# Autodesk Inventor assembly: PortaPiezas
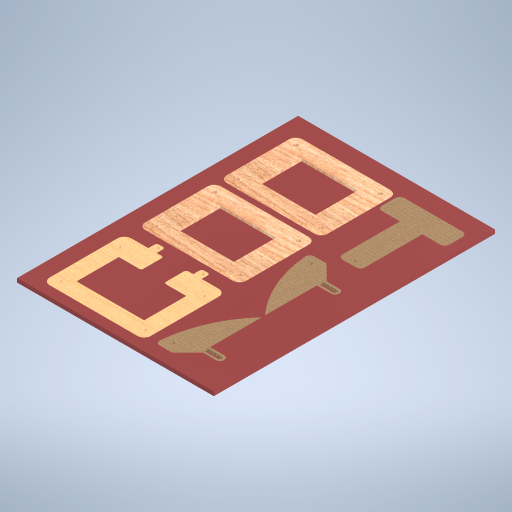
[picture p0: Inventor's stored thumbnail of the model, 512x512]
Saved by Autodesk Inventor 2023.1 (Build 271208000, 208)
## iProperties
Created: 2022-11-11
Part Number: PortaPiezas
Document SubType Name: Assembly
Designer: Daniel Peña
Author: Daniel Peña
## Documents named in this file (8)
- C:\Users\danie\Documents\UN\ProyectoRobotica\CAD\V3 - BigChungus\PortaPiezas.iam
- C:\Users\danie\Documents\UN\ProyectoRobotica\CAD\V3 - BigChungus\Base.ipt
- C:\Users\danie\Documents\UN\ProyectoRobotica\CAD\V3 - BigChungus\MarcoRompecabezas.ipt
- C:\Users\danie\Documents\UN\ProyectoRobotica\CAD\V3 - BigChungus\MarcoBC.ipt
- C:\Users\danie\Documents\UN\ProyectoRobotica\CAD\V3 - BigChungus\PistonBC.ipt
- C:\Users\danie\Documents\UN\ProyectoRobotica\CAD\V3 - BigChungus\TapaBC.ipt
- C:\Users\danie\Documents\UN\ProyectoRobotica\CAD\V3 - BigChungus\Dedo-BC.ipt
- C:\Users\danie\Documents\UN\ProyectoRobotica\CAD\PortaHerramienta\Ventosa.ipt
## Components (9 placed, 7 different names)
1. Base:1 — Flush:1, Mate:13, Mate:14, Mate:15, Mate:16, Mate:17, Mate:18, Flush:2, Flush:3
2. MarcoRompecabezas:1 — Flush:1, Mate:19, Flush:2, Flush:3, Mate:20, Mate:21, Mate:22, Mate:23, Mate:24, Mate:25, Mate:26, Mate:27, Mate:28, Mate:29, Mate:30, Mate:31
3. MarcoBC:1 — Mate:13, Mate:24, Mate:25
4. PistonBC:1 — Mate:16, Mate:30, Mate:31
5. TapaBC:1 — Mate:14, Mate:26, Mate:27
6. TapaBC:2 — Mate:15, Mate:28, Mate:29
7. Dedo-BC:1 — Mate:18, Mate:20, Mate:21
8. Dedo-BC:2 — Mate:17, Mate:22, Mate:23
9. Ventosa:1 — Mate:19
## Relationships (22: Mate 19, Flush 3)
- Flush:1: Base:1 ↔ MarcoRompecabezas:1
- Mate:13: Base:1 ↔ MarcoBC:1
- Mate:14: Base:1 ↔ TapaBC:1
- Mate:15: Base:1 ↔ TapaBC:2
- Mate:16: Base:1 ↔ PistonBC:1
- Mate:17: Base:1 ↔ Dedo-BC:2
- Mate:18: Base:1 ↔ Dedo-BC:1
- Mate:19: MarcoRompecabezas:1 ↔ Ventosa:1
- Flush:2: Base:1 ↔ MarcoRompecabezas:1
- Flush:3: Base:1 ↔ MarcoRompecabezas:1
- Mate:20: MarcoRompecabezas:1 ↔ Dedo-BC:1
- Mate:21: MarcoRompecabezas:1 ↔ Dedo-BC:1
- Mate:22: MarcoRompecabezas:1 ↔ Dedo-BC:2
- Mate:23: MarcoRompecabezas:1 ↔ Dedo-BC:2
- Mate:24: MarcoRompecabezas:1 ↔ MarcoBC:1
- Mate:25: MarcoRompecabezas:1 ↔ MarcoBC:1
- Mate:26: MarcoRompecabezas:1 ↔ TapaBC:1
- Mate:27: MarcoRompecabezas:1 ↔ TapaBC:1
- Mate:28: MarcoRompecabezas:1 ↔ TapaBC:2
- Mate:29: MarcoRompecabezas:1 ↔ TapaBC:2
- Mate:30: MarcoRompecabezas:1 ↔ PistonBC:1
- Mate:31: MarcoRompecabezas:1 ↔ PistonBC:1
